# Autodesk Inventor assembly: Chain Drive
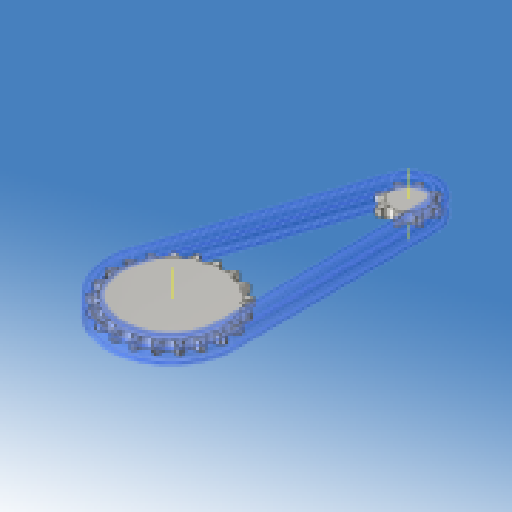
[picture p0: Inventor's stored thumbnail of the model, 512x512]
Saved by Autodesk Inventor 2024 (Build 280153000, 153)
## iProperties
ClientObjectVersion: 1
Created: 2024-02-29
Part Number: Chain Drive
Document SubType Name: Assembly
Designer: seene
Author: seene
## Documents named in this file (3)
- C:\Users\seene\OneDrive\SBRT\Robocup Rescue\Drive\RCR_drive\Design Accelerator\Chain Drive1.iam
- C:\Users\seene\OneDrive\SBRT\Robocup Rescue\Drive\RCR_drive\Design Accelerator\Roller Chain1.ipt
- C:\Users\seene\OneDrive\SBRT\Robocup Rescue\Drive\RCR_drive\Design Accelerator\Roller Chain Sprocket21.ipt
## Components (2 placed, 2 different names)
1. Roller Chain:1 — Flush:1, Mate:1, Mate:2
2. Roller Chain Sprocket2:1 — Flush:1, Mate:1, Mate:2
## Relationships (3: Mate 2, Flush 1)
- Flush:1: Roller Chain:1 ↔ Roller Chain Sprocket2:1
- Mate:1: Roller Chain:1 ↔ Roller Chain Sprocket2:1
- Mate:2: Roller Chain:1 ↔ Roller Chain Sprocket2:1
